# Autodesk Inventor assembly: X-AXIS ASSEMBLY
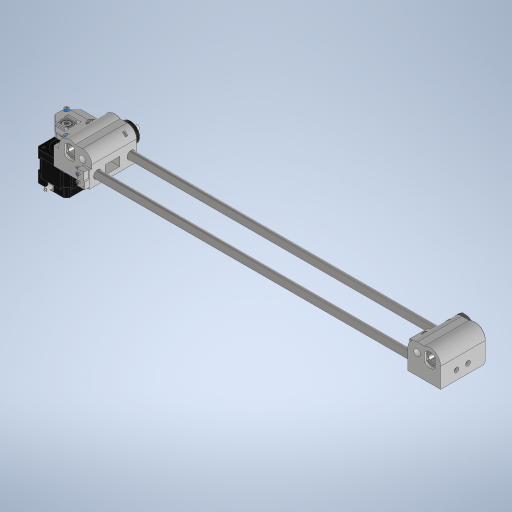
[picture p0: Inventor's stored thumbnail of the model, 512x512]
Saved by Autodesk Inventor 2023 (Build 270158000, 158)
## iProperties
Created: 2019-09-17
Part Number: X-AXIS ASSEMBLY
Document SubType Name: Assembly
Designer: pepd9
Mass: 1032.66 g
Surface Area: 1409.93 cm^2
Volume: 333.666 cm^3
Density: 3.0949 g/cm^3
Author: pepd9
## Documents named in this file (5)
- D:\000 - PEPCORP CLOUD\00- Legacy\Designs\MK3PRO P1\X-Axis\X-AXIS ASSEMBLY.iam
- D:\000 - PEPCORP CLOUD\00- Legacy\Designs\MK3PRO P1\X-Axis\X-AXIS ROD.ipt
- D:\000 - PEPCORP CLOUD\00- Legacy\Designs\MK3PRO P1\COMPONENTS\Small Limit Switch.iam
- D:\000 - PEPCORP CLOUD\00- Legacy\Designs\MK3PRO P1\X-Axis\X-End-Motor v0.3.iam
- D:\000 - PEPCORP CLOUD\00- Legacy\Designs\MK3PRO P1\X-Axis\X-End-Idler v0.1.iam
## Components (5 placed, 4 different names)
1. X-AXIS ROD:1 — Mate:123, Mate:124, Mate:125
2. X-AXIS ROD:2 — Mate:118, Mate:120
3. Small Limit Switch:1 [sub-assembly]
4. X-End-Motor v0.3:1 [sub-assembly] — Mate:118, Mate:122, Mate:124, Mate:125
5. X-End-Idler v0.1:1 [sub-assembly] — Mate:120, Mate:122, Mate:123
## Relationships (6: Mate 6)
- Mate:118: X-AXIS ROD:2 ↔ X-End-Motor v0.3:1
- Mate:120: X-AXIS ROD:2 ↔ X-End-Idler v0.1:1
- Mate:122 (450 mm): X-End-Motor v0.3:1 ↔ X-End-Idler v0.1:1
- Mate:123: X-AXIS ROD:1 ↔ X-End-Idler v0.1:1
- Mate:124: X-AXIS ROD:1 ↔ X-End-Motor v0.3:1
- Mate:125: X-AXIS ROD:1 ↔ X-End-Motor v0.3:1
